# Autodesk Inventor assembly: Assembly1
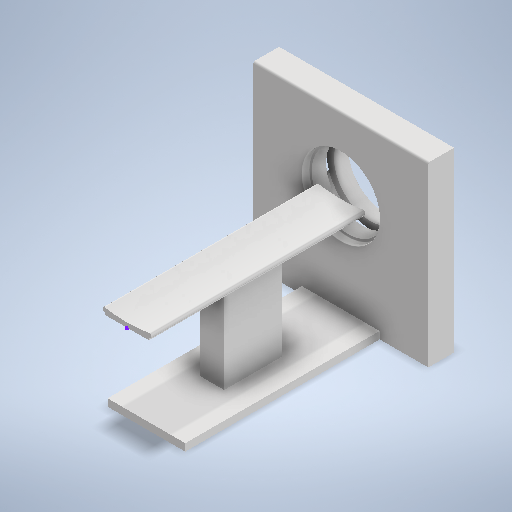
[picture p0: Inventor's stored thumbnail of the model, 512x512]
Saved by Autodesk Inventor 2025.2 (Build 292293000, 293)
## iProperties
Created: 2025-04-14
Part Number: Assembly1
Document SubType Name: Assembly
Designer: zenithprime
Author: zenithprime
## Documents named in this file (5)
- W:\Random Stuff\Coursework\Semester 6\ME 337 - Mechanical Systems Design\Assembly1.iam
- W:\Random Stuff\Coursework\Semester 6\ME 337 - Mechanical Systems Design\Gantry mssd.ipt
- W:\Random Stuff\Coursework\Semester 6\ME 337 - Mechanical Systems Design\Source.ipt
- W:\Random Stuff\Coursework\Semester 6\ME 337 - Mechanical Systems Design\source holder.ipt
- W:\Random Stuff\Coursework\Semester 6\ME 337 - Mechanical Systems Design\Patient_table\Patient_table\Patient_table.ipt
## Components (4 placed, 4 different names)
1. Gantry mssd:1 — Mate:4, Mate:5, Mate:6, Rotational:1
2. Source:1 — Mate:1, Mate:2, Mate:3
3. source holder:1 — Mate:1, Mate:2, Mate:3, Rotational:1
4. Patient_table:1 — Mate:4, Mate:5, Mate:6
## Relationships (7: Mate 6, RevoluteJoint 1)
- Mate:1: Source:1 ↔ source holder:1
- Mate:2: Source:1 ↔ source holder:1
- Mate:3: Source:1 ↔ source holder:1
- Mate:4: Gantry mssd:1 ↔ Patient_table:1
- Mate:5: Gantry mssd:1 ↔ Patient_table:1
- Mate:6: Gantry mssd:1 ↔ Patient_table:1
- Rotational:1 [RevoluteJoint] (8 mm): Gantry mssd:1 ↔ source holder:1
